# Autodesk Inventor assembly: scraper
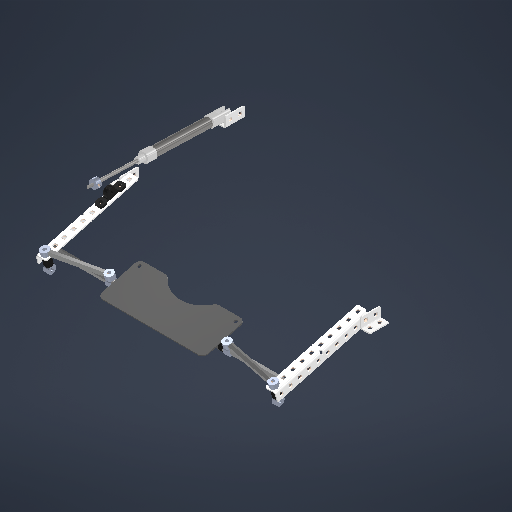
[picture p0: Inventor's stored thumbnail of the model, 512x512]
Saved by Autodesk Inventor 2025.2 (Build 292293000, 293)
## iProperties
Created: 2025-12-09
Part Number: scraper
Document SubType Name: Assembly
Designer: cloudy
Author: cloudy
## Documents named in this file (18)
- C:\Users\cloudy\Documents\GitHub\aura-cad\15\scraper.iam
- C:\Users\cloudy\Documents\GitHub\aura-cad\!lib\Structure\C Channel\Aluminum 1x3x1 Half\Alu C Half 1x3x1x2.ipt
- C:\Users\cloudy\Documents\GitHub\aura-cad\!lib\Structure\Standoff.ipt
- C:\Users\cloudy\Documents\GitHub\aura-cad\15\match_loader.ipt
- C:\Users\cloudy\Documents\GitHub\aura-cad\!lib\Structure\Standoff\Standoff 2.50.ipt
- C:\Users\cloudy\Documents\GitHub\aura-cad\!lib\Motion\Shaft LS\Shaft Collar Metal\Shaft Collar No Screw.iam
- C:\Users\cloudy\Documents\GitHub\aura-cad\!lib\Motion\Shaft LS\Shaft Collar Metal.iam
- C:\Users\cloudy\Documents\GitHub\aura-cad\!lib\Structure\Standoff\Standoff 3.00.ipt
- C:\Users\cloudy\Documents\GitHub\aura-cad\!lib\Motion\Spacers\Spacer Nylon .375 OD\NSpacer .375 OD x .250.ipt
- C:\Users\cloudy\Documents\GitHub\aura-cad\!lib\Motion\Spacers\Spacer Nylon .375 OD.ipt
- C:\Users\cloudy\Documents\GitHub\aura-cad\!lib\Motion\Spacers\Washer Steel\SWasher .375 OD x .062500.ipt
- C:\Users\cloudy\Documents\GitHub\aura-cad\!lib\Motion\Spacers\Washer Steel.ipt
- C:\Users\cloudy\Documents\GitHub\aura-cad\!lib\Motion\Spacers\Spacer Nylon .375 OD\NSpacer .375 OD x .500.ipt
- C:\Users\cloudy\Documents\GitHub\aura-cad\!lib\Structure\Standoff\Standoff 4.00.ipt
- C:\Users\cloudy\Documents\GitHub\aura-cad\!lib\Motion\Spacers\Spacer Nylon .375 OD\NSpacer .375 OD x .375.ipt
- C:\Users\cloudy\Documents\GitHub\aura-cad\!lib\Motion\Shaft LS\LS Pillow Bearing Block.ipt
- C:\Users\cloudy\Documents\GitHub\aura-cad\!lib\Motion\Pneumatics\Legacy - SMC Pneumatics\Double Acting Piston.iam
- C:\Users\cloudy\Documents\GitHub\aura-cad\!lib\Structure\C Channel\Aluminum 1x3x1 Half\Alu C Half 1x3x1x10.ipt
## Components (30 placed, 13 different names)
1. Alu C Half 1x3x1x2:1 — Mate:1, Flush:1, Mate:2, Flush:3, Flush:2, Mate:11, Insert:36
2. Alu C Half 1x3x1x2:2 — Mate:1, Flush:1, Mate:2, Insert:10
3. Alu C Half 1x3x1x10:1 — Insert:10, Insert:20, Insert:21, Angle:1, Insert:25, Insert:26, Angle:3
4. match_loader:1 — Insert:30, Angle:3, Insert:34, Insert:35
5. Standoff 3.00:1 — Insert:11
6. Shaft Collar No Screw:1 [sub-assembly] — Insert:11, Mate:4, Insert:15
7. Shaft Collar No Screw:2 [sub-assembly] — Mate:5, Insert:38
8. Shaft Collar No Screw:3 [sub-assembly] — Mate:4, Mate:5, Insert:13, Flush:4
9. Standoff 2.50:2 — Insert:13
10. NSpacer .375 OD x .250:1 — Insert:14, Insert:34
11. SWasher .375 OD x .062500:1 — Insert:14, Insert:15
12. Standoff 3.00:3 — Insert:20
13. Shaft Collar No Screw:4 [sub-assembly] — Angle:1, Mate:6
14. Shaft Collar No Screw:5 [sub-assembly] — Insert:21, Mate:7
15. NSpacer .375 OD x .250:2 — Insert:35
16. SWasher .375 OD x .062500:2
17. Standoff 2.50:5 — Insert:23, Mate:7
18. Shaft Collar No Screw:6 [sub-assembly] — Insert:23, Mate:6, Flush:4
19. Shaft Collar No Screw:7 [sub-assembly] — Insert:40
20. Shaft Collar No Screw:8 [sub-assembly] — Insert:25
21. NSpacer .375 OD x .500:3 — Insert:39, Insert:40
22. NSpacer .375 OD x .500:4 — Insert:26
23. Standoff 4.00:6 — Insert:28, Insert:29
24. NSpacer .375 OD x .375:5 — Insert:28
25. NSpacer .375 OD x .375:6 — Insert:29, Insert:30
26. LS Pillow Bearing Block:1 — Mate:9, Insert:37, Mate:12
27. Double Acting Piston:1 [sub-assembly] — Insert:32, Insert:33
28. Shaft Collar No Screw:9 [sub-assembly] — Insert:32, Mate:9
29. Alu C Half 1x3x1x2:3 — Insert:33, Flush:3, Flush:2, Mate:11
30. Alu C Half 1x3x1x10:2 — Insert:36, Insert:37, Mate:12, Insert:38, Insert:39
## Relationships (40: Insert 25, Mate 9, Flush 4, Angle 2)
- Mate:1: Alu C Half 1x3x1x2:1 ↔ Alu C Half 1x3x1x2:2
- Flush:1: Alu C Half 1x3x1x2:1 ↔ Alu C Half 1x3x1x2:2
- Mate:2 (330.2 mm): Alu C Half 1x3x1x2:1 ↔ Alu C Half 1x3x1x2:2
- Insert:10: Alu C Half 1x3x1x2:2 ↔ Alu C Half 1x3x1x10:1
- Insert:11: Standoff 3.00:1 ↔ Shaft Collar No Screw:1
- Mate:4: Shaft Collar No Screw:1 ↔ Shaft Collar No Screw:3
- Mate:5: Shaft Collar No Screw:2 ↔ Shaft Collar No Screw:3
- Insert:13: Shaft Collar No Screw:3 ↔ Standoff 2.50:2
- Insert:14: NSpacer .375 OD x .250:1 ↔ SWasher .375 OD x .062500:1
- Insert:15: Shaft Collar No Screw:1 ↔ SWasher .375 OD x .062500:1
- [Insert]: Standoff 3.00:3 ↔ Shaft Collar No Screw:4
- [Insert]: NSpacer .375 OD x .250:2 ↔ SWasher .375 OD x .062500:2
- [Insert]: Shaft Collar No Screw:4 ↔ SWasher .375 OD x .062500:2
- Insert:20: Alu C Half 1x3x1x10:1 ↔ Standoff 3.00:3
- Insert:21: Alu C Half 1x3x1x10:1 ↔ Shaft Collar No Screw:5
- Angle:1 (180 deg): Alu C Half 1x3x1x10:1 ↔ Shaft Collar No Screw:4
- Insert:23: Standoff 2.50:5 ↔ Shaft Collar No Screw:6
- Mate:6: Shaft Collar No Screw:4 ↔ Shaft Collar No Screw:6
- Mate:7: Shaft Collar No Screw:5 ↔ Standoff 2.50:5
- Insert:25 (12.7 mm): Alu C Half 1x3x1x10:1 ↔ Shaft Collar No Screw:8
- Insert:26: Alu C Half 1x3x1x10:1 ↔ NSpacer .375 OD x .500:4
- Insert:28: Standoff 4.00:6 ↔ NSpacer .375 OD x .375:5
- Insert:29: Standoff 4.00:6 ↔ NSpacer .375 OD x .375:6
- Insert:30: match_loader:1 ↔ NSpacer .375 OD x .375:6
- Insert:32 (7 mm): Double Acting Piston:1 ↔ Shaft Collar No Screw:9
- Mate:9: LS Pillow Bearing Block:1 ↔ Shaft Collar No Screw:9
- Insert:33 (3.175 mm): Double Acting Piston:1 ↔ Alu C Half 1x3x1x2:3
- Flush:3: Alu C Half 1x3x1x2:1 ↔ Alu C Half 1x3x1x2:3
- Flush:2: Alu C Half 1x3x1x2:1 ↔ Alu C Half 1x3x1x2:3
- Flush:4: Shaft Collar No Screw:3 ↔ Shaft Collar No Screw:6
- Mate:11 (127 mm): Alu C Half 1x3x1x2:1 ↔ Alu C Half 1x3x1x2:3
- Angle:3 (0 deg): Alu C Half 1x3x1x10:1 ↔ match_loader:1
- Insert:34: match_loader:1 ↔ NSpacer .375 OD x .250:1
- Insert:35: match_loader:1 ↔ NSpacer .375 OD x .250:2
- Insert:36: Alu C Half 1x3x1x2:1 ↔ Alu C Half 1x3x1x10:2
- Insert:37: LS Pillow Bearing Block:1 ↔ Alu C Half 1x3x1x10:2
- Mate:12: LS Pillow Bearing Block:1 ↔ Alu C Half 1x3x1x10:2
- Insert:38: Shaft Collar No Screw:2 ↔ Alu C Half 1x3x1x10:2
- Insert:39: NSpacer .375 OD x .500:3 ↔ Alu C Half 1x3x1x10:2
- Insert:40: Shaft Collar No Screw:7 ↔ NSpacer .375 OD x .500:3
## Named parameters: d28_d24 = 0 mm, d29_d25 = 0 mm, d30_d19 = 0 mm
